# Autodesk Inventor assembly: HS 84T Gear, Circle_MIR
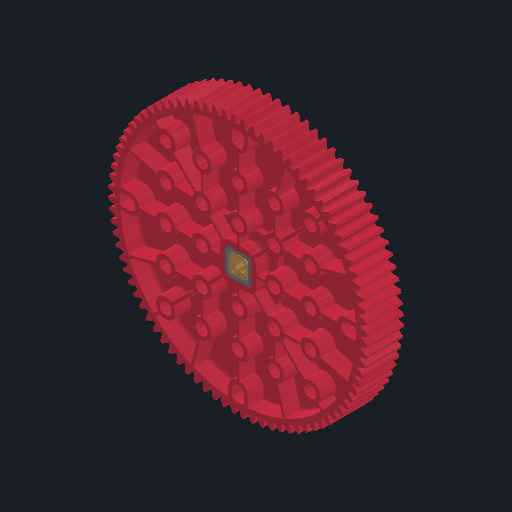
[picture p0: Inventor's stored thumbnail of the model, 512x512]
Saved by Autodesk Inventor 2024 (Build 280153000, 153)
## iProperties
Created: 2022-08-02
Part Number: HS 84T Gear, Circle_MIR
Document SubType Name: Assembly
Designer: macbook
Author: ylu12
## Documents named in this file (3)
- \\Mac\Home\Desktop\code\7899V-VRC-OVER-UNDER\Cad\VEX-CAD-Inventor-1.4.0\Motion\Gears\HS Gear\HS 84T Gear, Circle_MIR.iam
- \\Mac\Home\Desktop\code\7899V-VRC-OVER-UNDER\Cad\VEX-CAD-Inventor-1.4.0\Motion\HS Shaft Adapter Circle_MIR.ipt
- \\Mac\Home\Desktop\code\7899V-VRC-OVER-UNDER\Cad\VEX-CAD-Inventor-1.4.0\Motion\Gears\Reference Files\HS 84T Gear, No Insert_MIR.ipt
## Components (2 placed, 2 different names)
1. HS Shaft Adapter Circle_MIR:1 — Flush:1, Mate:2, Mate:1
2. HS 84T Gear, No Insert_MIR:1 — Mate:18, Mate:17, Flush:9
## Relationships (6: Mate 4, Flush 2)
- Flush:1 (-6.35 mm): HS Shaft Adapter Circle_MIR:1
- Mate:2: HS Shaft Adapter Circle_MIR:1
- Mate:1: HS Shaft Adapter Circle_MIR:1
- Mate:18: HS 84T Gear, No Insert_MIR:1
- Mate:17: HS 84T Gear, No Insert_MIR:1
- Flush:9: HS 84T Gear, No Insert_MIR:1
